# Autodesk Inventor assembly: Double Sided Bolt Assembly
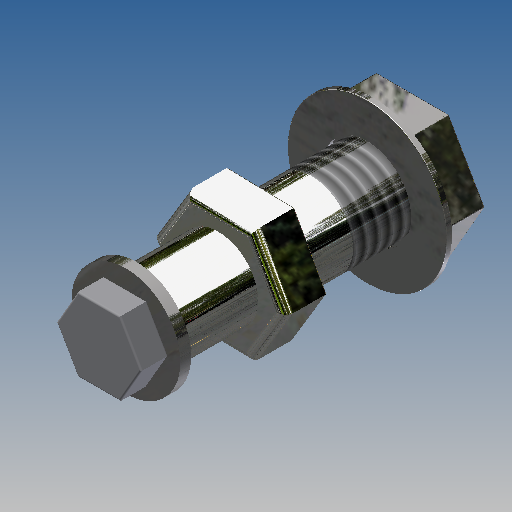
[picture p0: Inventor's stored thumbnail of the model, 512x512]
Saved by Autodesk Inventor 2018 (Build 220112000, 112)
## iProperties
Created: 2018-04-08
Part Number: Double Sided Bolt Assembly
Document SubType Name: Assembly
Designer: Cole
Author: Cole
## Documents named in this file (6)
- D:\Cole\Documents\GitHub\SchoolCAD\ReverseEngineering\Double Sided Bolt Assembly.iam
- D:\Cole\Documents\GitHub\SchoolCAD\ReverseEngineering\Double Sided Bolt.ipt
- D:\Cole\Documents\GitHub\SchoolCAD\ReverseEngineering\Small Bolt.ipt
- D:\Cole\Documents\GitHub\SchoolCAD\ReverseEngineering\Small Washer.ipt
- D:\Cole\Documents\GitHub\SchoolCAD\ReverseEngineering\Large Nut.ipt
- D:\Cole\Documents\GitHub\SchoolCAD\ReverseEngineering\Large Washer.ipt
## Components (5 placed, 5 different names)
1. Double Sided Bolt:1 — Insert:2, Insert:4
2. Small Bolt:1 — Insert:1
3. Small Washer:1 — Insert:1, Insert:2
4. Large Nut:1 — Insert:3, Insert:4
5. Large Washer:1 — Insert:3
## Relationships (4: Insert 4)
- Insert:1: Small Bolt:1 ↔ Small Washer:1
- Insert:2: Double Sided Bolt:1 ↔ Small Washer:1
- Insert:3: Large Nut:1 ↔ Large Washer:1
- Insert:4: Double Sided Bolt:1 ↔ Large Nut:1
